# Autodesk Inventor assembly: HbIndexMotorU01
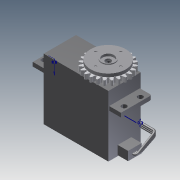
[picture p0: Inventor's stored thumbnail of the model, 180x180]
Saved by Autodesk Inventor 2015 SP1 (Build 190203100, 203)
## iProperties
Created: 2015-02-14
Part Number: HbIndexMotorU01
Document SubType Name: Assembly
Designer: Yamaura
Author: Yamaura
## Documents named in this file (5)
- C:\Users\Yamaura\Documents\GitHub\HACKberry\HACKberry-hardware\3D\Inventor\Parts\HbIndexMotorU01.iam
- C:\Users\Yamaura\Documents\GitHub\HACKberry\HACKberry-hardware\3D\Inventor\Parts\HbServoHorn01.ipt
- C:\Users\Yamaura\Documents\GitHub\HACKberry\HACKberry-hardware\3D\Inventor\Parts\HbIndexMotorGear02.ipt
- C:\Users\Yamaura\Documents\GitHub\HACKberry\HACKberry-hardware\3D\Inventor\Parts\GWS_S03N.ipt
- C:\Users\Yamaura\Documents\GitHub\HACKberry\HACKberry-hardware\3D\Inventor\Parts\flatScrewM2L6PHI3.3T1.3.ipt
## Components (7 placed, 4 different names)
1. GWS_S03N:1 — メイト:1, フラッシュ:1, フラッシュ:2
2. HbServoHorn01:1 — メイト:2, メイト:3, メイト:4, メイト:5, メイト:6, メイト:7, メイト:8
3. HbIndexMotorGear02:1 — メイト:5, メイト:6, メイト:7, フラッシュ:3
4. flatScrewM2L6PHI3.3T1.3:1 — メイト:8, フラッシュ:3
5. flatScrewM2L6PHI3.3T1.3:2
6. flatScrewM2L6PHI3.3T1.3:3
7. flatScrewM2L6PHI3.3T1.3:4
## Component patterns: (4 elements, first: flatScrewM2L6PHI3.3T1.3:1)
## Relationships (11: Mate 8, Flush 3)
- メイト:1 [Mate]: GWS_S03N:1
- フラッシュ:1 [Flush]: GWS_S03N:1
- フラッシュ:2 [Flush]: GWS_S03N:1
- メイト:2 [Mate]: HbServoHorn01:1
- メイト:3 [Mate]: HbServoHorn01:1
- メイト:4 [Mate]: HbServoHorn01:1
- メイト:5 [Mate]: HbServoHorn01:1 ↔ HbIndexMotorGear02:1
- メイト:6 [Mate]: HbServoHorn01:1 ↔ HbIndexMotorGear02:1
- メイト:7 [Mate]: HbServoHorn01:1 ↔ HbIndexMotorGear02:1
- メイト:8 [Mate]: HbServoHorn01:1 ↔ flatScrewM2L6PHI3.3T1.3:1
- フラッシュ:3 [Flush] (-1.3 mm): HbIndexMotorGear02:1 ↔ flatScrewM2L6PHI3.3T1.3:1
